# Autodesk Inventor assembly: Gripper_Arm
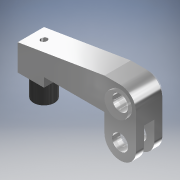
[picture p0: Inventor's stored thumbnail of the model, 180x180]
Saved by Autodesk Inventor 2021.3 (Build 253353000, 353)
## iProperties
Created: 2021-04-16
Part Number: Gripper_Arm
Document SubType Name: Assembly
Designer: domin
Author: domin
## Documents named in this file (5)
- E:\Transfer\Sync\Hivemind\1-MCI-Unterlagen\Master\Semester 2\Projekt 1\Hausberger\Workfolder_Dommy\Gripper\Gripper_Arm.iam
- E:\Transfer\Sync\Hivemind\1-MCI-Unterlagen\Master\Semester 2\Projekt 1\Hausberger\Workfolder_Dommy\Gripper\Gripper_Arm_Base.ipt
- E:\Transfer\Sync\Hivemind\1-MCI-Unterlagen\Master\Semester 2\Projekt 1\Hausberger\Workfolder_Dommy\Gripper\Zukauf\TFZF3-5.ipt
- E:\Transfer\Sync\Hivemind\1-MCI-Unterlagen\Master\Semester 2\Projekt 1\Hausberger\Workfolder_Dommy\Gripper\Zukauf\Gleitlager\TFZB3-3.ipt
- E:\Transfer\Sync\Hivemind\1-MCI-Unterlagen\Master\Semester 2\Projekt 1\Hausberger\Workfolder_Dommy\Gripper\Zukauf\251501403.ipt
## Components (6 placed, 4 different names)
1. Gripper_Arm_Base:1 — Mate:1, Mate:2, Mate:3, Mate:4, Mate:5, Mate:6, Mate:7, Mate:10, Mate:11, Flush:1, Flush:2, Mate:12, Mate:13, Angle:1
2. TFZF3-5:1 — Mate:5, Mate:7, Mate:8
3. TFZF3-5:2 — Mate:4, Mate:6, Mate:9
4. TFZB3-3:1 — Mate:10, Flush:1, Flush:3
5. TFZB3-3:2 — Mate:11, Flush:2, Flush:4
6. 251501403:1 — Mate:12, Mate:13, Angle:1
## Relationships (18: Mate 13, Flush 4, Angle 1)
- Mate:1: Gripper_Arm_Base:1
- Mate:2: Gripper_Arm_Base:1
- Mate:3: Gripper_Arm_Base:1
- Mate:4: Gripper_Arm_Base:1 ↔ TFZF3-5:2
- Mate:5: Gripper_Arm_Base:1 ↔ TFZF3-5:1
- Mate:6: Gripper_Arm_Base:1 ↔ TFZF3-5:2
- Mate:7: Gripper_Arm_Base:1 ↔ TFZF3-5:1
- Mate:8: TFZF3-5:1
- Mate:9: TFZF3-5:2
- Mate:10: Gripper_Arm_Base:1 ↔ TFZB3-3:1
- Mate:11: Gripper_Arm_Base:1 ↔ TFZB3-3:2
- Flush:1: Gripper_Arm_Base:1 ↔ TFZB3-3:1
- Flush:2: Gripper_Arm_Base:1 ↔ TFZB3-3:2
- Flush:3: TFZB3-3:1
- Flush:4: TFZB3-3:2
- Mate:12: Gripper_Arm_Base:1 ↔ 251501403:1
- Mate:13: Gripper_Arm_Base:1 ↔ 251501403:1
- Angle:1 (0 deg): Gripper_Arm_Base:1 ↔ 251501403:1
